# Autodesk Inventor assembly: ASY PNS-0110 frame left floor
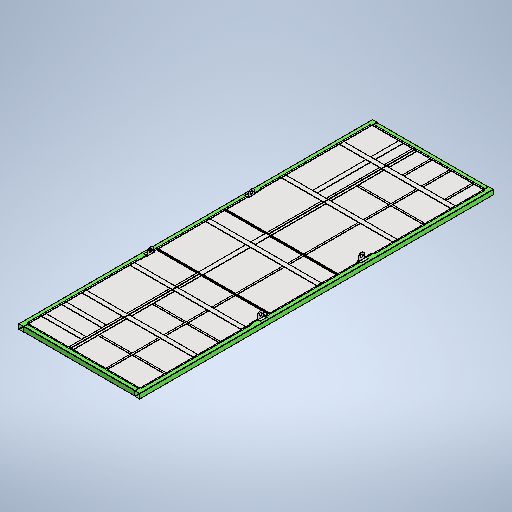
[picture p0: Inventor's stored thumbnail of the model, 512x512]
Saved by Autodesk Inventor 2025.1 (Build 291241020, 241B)
## iProperties
Created: 2025-03-10
Part Number: ASY PNS-0110 frame left floor
Document SubType Name: Assembly
Designer: admin
_SolveAssemblyDoc: Frame Generator Solve Assembly
_Version: 25.0.0
Author: admin
## Documents named in this file (11)
- C:\Users\user\YandexDisk-badmisterfox\home pc\Inventor\PNS-Panaevsk\ASY PNS-0110 frame left floor.iam
- C:\Users\user\YandexDisk-badmisterfox\home pc\Inventor\PNS-Panaevsk\PNS-0110 frame left floor.ipt
- C:\Users\user\YandexDisk-badmisterfox\home pc\Inventor\PNS-Panaevsk\ASY PNS-0110 frame left floor\Frame\Frame 1741580713954.iam
- C:\Users\user\YandexDisk-badmisterfox\home pc\Inventor\PNS-Panaevsk\PNS-0111 floor sheet 1.ipt
- C:\Users\user\YandexDisk-badmisterfox\home pc\Inventor\PNS-Panaevsk\PNS-0113 floor sheet 31.ipt
- C:\Users\user\YandexDisk-badmisterfox\home pc\Inventor\PNS-Panaevsk\PNS-0810 floor ring.ipt
- C:\Users\user\YandexDisk-badmisterfox\home pc\Inventor\PNS-Panaevsk\PNS-0812 floor ring  strengthen.ipt
- C:\Users\user\YandexDisk-badmisterfox\home pc\Inventor\PNS-Panaevsk\PNS-0114 floor sheet 41.ipt
- C:\Users\user\YandexDisk-badmisterfox\home pc\Inventor\PNS-Panaevsk\PNS-0115 floor sheet 5.ipt
- C:\Users\user\YandexDisk-badmisterfox\home pc\Inventor\PNS-Panaevsk\PNS-0116 floor sheet 6.ipt
- C:\Users\user\YandexDisk-badmisterfox\home pc\Inventor\PNS-Panaevsk\PNS-0111 floor sheet 2_CPY.ipt
## Components (16 placed, 10 different names)
1. PNS-0110 frame left floor:1
2. Frame 1741580713954:1 [sub-assembly] — Rigid:1, Mate:1, Flush:1, Flush:2, Mate:10, Mate:11, Mate:12, Mate:13, Mate:14, Mate:15, Mate:16, Mate:17, Flush:5, Flush:6, Mate:18, Flush:7, Flush:8, Mate:19, Flush:9, Flush:10, Mate:20, Mate:22, Flush:12, Flush:13
3. PNS-0111 floor sheet 1:1 — Rigid:1
4. PNS-0113 floor sheet 3:2 — Mate:1, Flush:1, Flush:2
5. PNS-0810 floor ring:1
6. PNS-0812 floor ring  strengthen:1 — Mate:10, Mate:11, Flush:3, Flush:5
7. PNS-0810 floor ring:2
8. PNS-0812 floor ring  strengthen:2 — Mate:12, Mate:13, Flush:4, Flush:6
9. PNS-0810 floor ring:3
10. PNS-0812 floor ring  strengthen:3 — Mate:14, Mate:15, Flush:4
11. PNS-0810 floor ring:4
12. PNS-0812 floor ring  strengthen:4 — Mate:16, Mate:17, Flush:3
13. PNS-0114 floor sheet 41:1 — Mate:18, Flush:7, Flush:8, Flush:11, Mate:21
14. PNS-0115 floor sheet 5:1 — Mate:19, Flush:9, Flush:10
15. PNS-0116 floor sheet 6:1 — Mate:20, Flush:11, Mate:21
16. PNS-0117 floor sheet 7:1 — Mate:22, Flush:12, Flush:13
## Relationships (40: Mate 22, Flush 13, Tangent 4, WeldJoint 1)
- Rigid:1 [WeldJoint]: Frame 1741580713954:1 ↔ PNS-0111 floor sheet 1:1
- Mate:1: Frame 1741580713954:1 ↔ PNS-0113 floor sheet 3:2
- Flush:1 (70 mm): Frame 1741580713954:1 ↔ PNS-0113 floor sheet 3:2
- Flush:2 (70 mm): Frame 1741580713954:1 ↔ PNS-0113 floor sheet 3:2
- [Mate]: PNS-0810 floor ring:1 ↔ PNS-0812 floor ring  strengthen:1
- [Mate]: PNS-0810 floor ring:1 ↔ PNS-0812 floor ring  strengthen:1
- [Tangent] (20 mm): PNS-0810 floor ring:1 ↔ PNS-0812 floor ring  strengthen:1
- [Mate]: PNS-0810 floor ring:2 ↔ PNS-0812 floor ring  strengthen:2
- [Mate]: PNS-0810 floor ring:2 ↔ PNS-0812 floor ring  strengthen:2
- [Tangent] (20 mm): PNS-0810 floor ring:2 ↔ PNS-0812 floor ring  strengthen:2
- [Mate]: PNS-0810 floor ring:3 ↔ PNS-0812 floor ring  strengthen:3
- [Mate]: PNS-0810 floor ring:3 ↔ PNS-0812 floor ring  strengthen:3
- [Tangent] (20 mm): PNS-0810 floor ring:3 ↔ PNS-0812 floor ring  strengthen:3
- [Mate]: PNS-0810 floor ring:4 ↔ PNS-0812 floor ring  strengthen:4
- [Mate]: PNS-0810 floor ring:4 ↔ PNS-0812 floor ring  strengthen:4
- [Tangent] (20 mm): PNS-0810 floor ring:4 ↔ PNS-0812 floor ring  strengthen:4
- Mate:10: Frame 1741580713954:1 ↔ PNS-0812 floor ring  strengthen:1
- Mate:11: Frame 1741580713954:1 ↔ PNS-0812 floor ring  strengthen:1
- Mate:12: Frame 1741580713954:1 ↔ PNS-0812 floor ring  strengthen:2
- Mate:13: Frame 1741580713954:1 ↔ PNS-0812 floor ring  strengthen:2
- Mate:14: Frame 1741580713954:1 ↔ PNS-0812 floor ring  strengthen:3
- Mate:15: Frame 1741580713954:1 ↔ PNS-0812 floor ring  strengthen:3
- Mate:16: Frame 1741580713954:1 ↔ PNS-0812 floor ring  strengthen:4
- Mate:17: Frame 1741580713954:1 ↔ PNS-0812 floor ring  strengthen:4
- Flush:3: PNS-0812 floor ring  strengthen:1 ↔ PNS-0812 floor ring  strengthen:4
- Flush:4: PNS-0812 floor ring  strengthen:2 ↔ PNS-0812 floor ring  strengthen:3
- Flush:5 (2430 mm): Frame 1741580713954:1 ↔ PNS-0812 floor ring  strengthen:1
- Flush:6 (2430 mm): Frame 1741580713954:1 ↔ PNS-0812 floor ring  strengthen:2
- Mate:18: Frame 1741580713954:1 ↔ PNS-0114 floor sheet 41:1
- Flush:7 (70 mm): Frame 1741580713954:1 ↔ PNS-0114 floor sheet 41:1
- Flush:8 (70 mm): Frame 1741580713954:1 ↔ PNS-0114 floor sheet 41:1
- Mate:19: Frame 1741580713954:1 ↔ PNS-0115 floor sheet 5:1
- Flush:9 (70 mm): Frame 1741580713954:1 ↔ PNS-0115 floor sheet 5:1
- Flush:10 (70 mm): Frame 1741580713954:1 ↔ PNS-0115 floor sheet 5:1
- Mate:20: Frame 1741580713954:1 ↔ PNS-0116 floor sheet 6:1
- Flush:11: PNS-0114 floor sheet 41:1 ↔ PNS-0116 floor sheet 6:1
- Mate:21 (10 mm): PNS-0114 floor sheet 41:1 ↔ PNS-0116 floor sheet 6:1
- Mate:22: Frame 1741580713954:1 ↔ PNS-0117 floor sheet 7:1
- Flush:12 (70 mm): Frame 1741580713954:1 ↔ PNS-0117 floor sheet 7:1
- Flush:13 (70 mm): Frame 1741580713954:1 ↔ PNS-0117 floor sheet 7:1
## Named parameters: d101_d95_d68_d63_d62 = 0 mm, d102_d96_d69_d66 = 0 mm, d103_d97_d72 = 20 mm, d18_d101_d95_d68_d63_d62 = 0 mm, d19_d102_d96_d69_d66 = 0 mm, d20_d103_d97_d72 = 20 mm, d21_d101_d95_d68_d63_d62 = 0 mm, d22_d102_d96_d69_d66 = 0 mm, d23_d103_d97_d72 = 20 mm, d24_d101_d95_d68_d63_d62 = 0 mm, d25_d102_d96_d69_d66 = 0 mm, d26_d103_d97_d72 = 20 mm
